# Autodesk Inventor assembly: YagiBoard
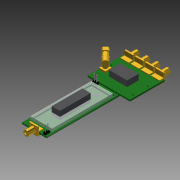
[picture p0: Inventor's stored thumbnail of the model, 180x180]
Saved by Autodesk Inventor 2014 (Build 180170000, 170)
## iProperties
Created: 2015-01-07
Part Number: YagiBoard
Document SubType Name: Assembly
Designer: Owner
Author: Owner
## Documents named in this file (11)
- C:\Users\Owner\Documents\APC\FrontEnd\IAM\Yagi\YagiBoard.iam
- C:\Users\Owner\Documents\APC\FrontEnd\IAM\Yagi\Yagi_Board.ipt
- C:\Users\Owner\Documents\APC\FrontEnd\IAM\Common\SMA_Edge.ipt
- C:\Users\Owner\Documents\APC\FrontEnd\IAM\Common\CombinerBoard.ipt
- C:\Users\Owner\Documents\APC\FrontEnd\IAM\Common\SMA_Up.ipt
- C:\Users\Owner\Documents\APC\FrontEnd\IAM\Common\SMA_RightAngle.ipt
- C:\Users\Owner\Documents\APC\FrontEnd\IAM\Common\4WayCombiner.ipt
- C:\Users\Owner\Documents\APC\FrontEnd\IAM\Common\BPF.ipt
- C:\Users\Owner\Documents\APC\FrontEnd\IAM\Common\FirstStageAmp.ipt
- C:\Users\Owner\Documents\APC\FrontEnd\IAM\Common\YagiCan.ipt
- C:\Users\Owner\Documents\APC\FrontEnd\IAM\Common\2PinHeader.ipt
## Components (15 placed, 10 different names)
1. Yagi_Board:1 — Mate:1, Mate:8, Flush:4, Mate:31, Mate:32, Flush:17, Flush:18, Flush:19, Flush:20, Flush:21, Flush:22, Flush:23, Flush:24, Flush:25, Mate:36, Mate:37, Flush:26, Flush:27, Flush:28, Flush:29, Flush:30
2. SMA_Edge:4 — Mate:1, Mate:8, Flush:4
3. CombinerBoard:1 — Mate:23, Mate:24, Mate:25, Mate:26, Mate:27, Mate:28, Mate:29, Mate:30, Flush:7, Flush:8, Flush:9, Flush:10, Mate:31, Mate:32, Mate:33, Flush:12, Flush:13, Angle:1, Flush:14, Flush:15, Flush:16, Flush:30
4. SMA_Edge:5 — Mate:26, Mate:29, Flush:9
5. SMA_Edge:6 — Mate:25, Mate:30, Flush:10
6. SMA_Edge:7 — Mate:24, Mate:27, Flush:8
7. SMA_Edge:8 — Mate:23, Mate:28, Flush:7
8. SMA_Up:1 — Mate:33, Flush:12, Flush:13, Mate:34, Mate:35
9. SMA_RightAngle:1 — Mate:34, Mate:35, Angle:1
10. 4WayCombiner:1 — Flush:14, Flush:15, Flush:16
11. BPF:1 — Flush:17, Flush:21, Flush:22
12. FirstStageAmp:1 — Flush:18, Flush:19, Flush:20
13. YagiCan:1 — Flush:23, Flush:24, Flush:25
14. 2PinHeader:1 — Mate:37, Flush:28, Flush:29
15. 2PinHeader:2 — Mate:36, Flush:26, Flush:27
## Relationships (42: Flush 24, Mate 17, Angle 1)
- Mate:1: Yagi_Board:1 ↔ SMA_Edge:4
- Mate:8: Yagi_Board:1 ↔ SMA_Edge:4
- Flush:4 (9.525 mm): Yagi_Board:1 ↔ SMA_Edge:4
- Mate:23: CombinerBoard:1 ↔ SMA_Edge:8
- Mate:24: CombinerBoard:1 ↔ SMA_Edge:7
- Mate:25: CombinerBoard:1 ↔ SMA_Edge:6
- Mate:26: CombinerBoard:1 ↔ SMA_Edge:5
- Mate:27: CombinerBoard:1 ↔ SMA_Edge:7
- Mate:28: CombinerBoard:1 ↔ SMA_Edge:8
- Mate:29: CombinerBoard:1 ↔ SMA_Edge:5
- Mate:30: CombinerBoard:1 ↔ SMA_Edge:6
- Flush:7 (-1.397 mm): CombinerBoard:1 ↔ SMA_Edge:8
- Flush:8 (12.827 mm): CombinerBoard:1 ↔ SMA_Edge:7
- Flush:9 (-24.257 mm): CombinerBoard:1 ↔ SMA_Edge:5
- Flush:10 (-35.687 mm): CombinerBoard:1 ↔ SMA_Edge:6
- Mate:31 (-3.175 mm): Yagi_Board:1 ↔ CombinerBoard:1
- Mate:32: Yagi_Board:1 ↔ CombinerBoard:1
- Mate:33: CombinerBoard:1 ↔ SMA_Up:1
- Flush:12 (11.8872 mm): CombinerBoard:1 ↔ SMA_Up:1
- Flush:13 (-0.8382 mm): CombinerBoard:1 ↔ SMA_Up:1
- Mate:34: SMA_Up:1 ↔ SMA_RightAngle:1
- Mate:35 (2 mm): SMA_Up:1 ↔ SMA_RightAngle:1
- Angle:1 (135 deg): CombinerBoard:1 ↔ SMA_RightAngle:1
- Flush:14: CombinerBoard:1 ↔ 4WayCombiner:1
- Flush:15 (12.9032 mm): CombinerBoard:1 ↔ 4WayCombiner:1
- Flush:16 (10.8204 mm): CombinerBoard:1 ↔ 4WayCombiner:1
- Flush:17: Yagi_Board:1 ↔ BPF:1
- Flush:18: Yagi_Board:1 ↔ FirstStageAmp:1
- Flush:19 (-10.6426 mm): Yagi_Board:1 ↔ FirstStageAmp:1
- Flush:20 (14.6558 mm): Yagi_Board:1 ↔ FirstStageAmp:1
- Flush:21 (8.6106 mm): Yagi_Board:1 ↔ BPF:1
- Flush:22 (25.8318 mm): Yagi_Board:1 ↔ BPF:1
- Flush:23: Yagi_Board:1 ↔ YagiCan:1
- Flush:24 (1.5494 mm): Yagi_Board:1 ↔ YagiCan:1
- Flush:25 (7.5184 mm): Yagi_Board:1 ↔ YagiCan:1
- Mate:36: Yagi_Board:1 ↔ 2PinHeader:2
- Mate:37: Yagi_Board:1 ↔ 2PinHeader:1
- Flush:26 (1.1176 mm): Yagi_Board:1 ↔ 2PinHeader:2
- Flush:27 (3.8608 mm): Yagi_Board:1 ↔ 2PinHeader:2
- Flush:28 (1.8288 mm): Yagi_Board:1 ↔ 2PinHeader:1
- Flush:29 (0.508 mm): Yagi_Board:1 ↔ 2PinHeader:1
- Flush:30 (-6.985 mm): Yagi_Board:1 ↔ CombinerBoard:1
